# Autodesk Inventor assembly: Catapult
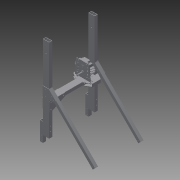
[picture p0: Inventor's stored thumbnail of the model, 180x180]
Saved by Autodesk Inventor 2013 (Build 170138000, 138)
## iProperties
Created: 2014-01-18
Part Number: Catapult
Document SubType Name: Assembly
Designer: 215152
Author: 215152
## Documents named in this file (9)
- E:\Robotics\FRC\2014\CAD\Robot\Catapult\Catapult.iam
- E:\Robotics\FRC\2014\CAD\Brian's Derp\Additions\SuperSuperStructure.ipt
- E:\Robotics\FRC\2014\CAD\Brian's Derp\Additions\CatapultGussetPlate.ipt
- E:\Robotics\FRC\2014\CAD\Brian's Derp\Additions\CatapultMotorSupport.ipt
- E:\Robotics\FRC\2014\CAD\Brian's Derp\Additions\SuperStructureSupport.ipt
- E:\Robotics\FRC\2014\CAD\Brian's Derp\Additions\SideSupport.ipt
- E:\Robotics\FRC\2014\CAD\Brian's Derp\Additions\SideGusset.ipt
- E:\Robotics\FRC\2014\CAD\Robot\Catapult\Structure\MotorSupport.ipt
- E:\Robotics\FRC\2014\CAD\Robot\Catapult\Structure\Imported Components\Toughbox-mini\Toughbox-mini.iam
## Components (16 placed, 8 different names)
1. SuperSuperStructure:1 — Mate:1, Flush:1, Flush:2, Mate:14, Flush:12, Mate:16, Mate:22, Flush:15, Mate:25, Flush:17, Mate:26
2. SuperSuperStructure:2 — Mate:1, Flush:1, Flush:2, Mate:13, Flush:11, Mate:15, Mate:21, Flush:14, Mate:23, Flush:16, Mate:24, Mate:27, Flush:21, Mate:36
3. CatapultGussetPlate:1 — Mate:34, Flush:25, Mate:35
4. CatapultGussetPlate:2 — Mate:28, Flush:22, Mate:29, Mate:40
5. CatapultGussetPlate:3 — Mate:32, Flush:24, Mate:33
6. CatapultGussetPlate:4 — Flush:23, Mate:30, Mate:31, Mate:36, Mate:41, Mate:42
7. CatapultMotorSupport:1 — Mate:27, Flush:21, Mate:28, Flush:22, Mate:29, Flush:23, Mate:30, Mate:31, Mate:32, Flush:24, Mate:33, Mate:34, Flush:25, Mate:35, Flush:26, Flush:27, Mate:44
8. SuperStructureSupport:1 — Mate:13, Flush:11, Mate:15
9. SuperStructureSupport:2 — Mate:14, Flush:12, Mate:16
10. SideSupport:1 — Mate:21, Flush:14, Flush:19
11. SideSupport:2 — Mate:22, Flush:15, Flush:20
12. SideGusset:1 — Mate:25, Flush:17, Mate:26, Flush:20
13. SideGusset:2 — Mate:23, Flush:16, Mate:24, Flush:19
14. MotorSupport:1 — Flush:26, Mate:41, Mate:42, Mate:43, Mate:45, Flush:28
15. MotorSupport:2 — Mate:40, Mate:43, Flush:27, Mate:46
16. Toughbox-mini:1 [sub-assembly] — Mate:44, Mate:45, Mate:46, Flush:28
## Relationships (46: Mate 28, Flush 18)
- Mate:1 (349.25 mm): SuperSuperStructure:1 ↔ SuperSuperStructure:2
- Flush:1: SuperSuperStructure:1 ↔ SuperSuperStructure:2
- Flush:2: SuperSuperStructure:1 ↔ SuperSuperStructure:2
- Mate:13: SuperSuperStructure:2 ↔ SuperStructureSupport:1
- Flush:11: SuperSuperStructure:2 ↔ SuperStructureSupport:1
- Mate:14: SuperSuperStructure:1 ↔ SuperStructureSupport:2
- Flush:12: SuperSuperStructure:1 ↔ SuperStructureSupport:2
- Mate:15: SuperSuperStructure:2 ↔ SuperStructureSupport:1
- Mate:16: SuperSuperStructure:1 ↔ SuperStructureSupport:2
- Mate:21: SuperSuperStructure:2 ↔ SideSupport:1
- Flush:14: SuperSuperStructure:2 ↔ SideSupport:1
- Mate:22: SuperSuperStructure:1 ↔ SideSupport:2
- Flush:15: SuperSuperStructure:1 ↔ SideSupport:2
- Mate:23: SuperSuperStructure:2 ↔ SideGusset:2
- Flush:16: SuperSuperStructure:2 ↔ SideGusset:2
- Mate:24: SuperSuperStructure:2 ↔ SideGusset:2
- Mate:25: SuperSuperStructure:1 ↔ SideGusset:1
- Flush:17: SuperSuperStructure:1 ↔ SideGusset:1
- Mate:26: SuperSuperStructure:1 ↔ SideGusset:1
- Flush:19: SideSupport:1 ↔ SideGusset:2
- Flush:20: SideSupport:2 ↔ SideGusset:1
- Mate:27: SuperSuperStructure:2 ↔ CatapultMotorSupport:1
- Flush:21: SuperSuperStructure:2 ↔ CatapultMotorSupport:1
- Mate:28: CatapultGussetPlate:2 ↔ CatapultMotorSupport:1
- Flush:22: CatapultGussetPlate:2 ↔ CatapultMotorSupport:1
- Mate:29: CatapultGussetPlate:2 ↔ CatapultMotorSupport:1
- Flush:23: CatapultGussetPlate:4 ↔ CatapultMotorSupport:1
- Mate:30: CatapultGussetPlate:4 ↔ CatapultMotorSupport:1
- Mate:31: CatapultGussetPlate:4 ↔ CatapultMotorSupport:1
- Mate:32: CatapultGussetPlate:3 ↔ CatapultMotorSupport:1
- Flush:24: CatapultGussetPlate:3 ↔ CatapultMotorSupport:1
- Mate:33: CatapultGussetPlate:3 ↔ CatapultMotorSupport:1
- Mate:34: CatapultGussetPlate:1 ↔ CatapultMotorSupport:1
- Flush:25: CatapultGussetPlate:1 ↔ CatapultMotorSupport:1
- Mate:35: CatapultGussetPlate:1 ↔ CatapultMotorSupport:1
- Mate:36 (-431.8 mm): SuperSuperStructure:2 ↔ CatapultGussetPlate:4
- Flush:26: CatapultMotorSupport:1 ↔ MotorSupport:1
- Mate:40: CatapultGussetPlate:2 ↔ MotorSupport:2
- Mate:41: CatapultGussetPlate:4 ↔ MotorSupport:1
- Mate:42: CatapultGussetPlate:4 ↔ MotorSupport:1
- Mate:43: MotorSupport:1 ↔ MotorSupport:2
- Flush:27: CatapultMotorSupport:1 ↔ MotorSupport:2
- Mate:44: CatapultMotorSupport:1 ↔ Toughbox-mini:1
- Mate:45 (3.175 mm): MotorSupport:1 ↔ Toughbox-mini:1
- Mate:46 (3.175 mm): MotorSupport:2 ↔ Toughbox-mini:1
- Flush:28 (-15.875 mm): MotorSupport:1 ↔ Toughbox-mini:1
